# Autodesk Inventor assembly: Vertical Support - with Brackets
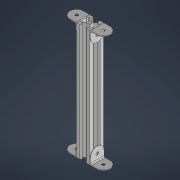
[picture p0: Inventor's stored thumbnail of the model, 180x180]
Saved by Autodesk Inventor 2022 (Build 260153000, 153)
## iProperties
Created: 2023-06-23
Part Number: Vertical Support - with Brackets
Document SubType Name: Assembly
Designer: Ryan Mitcham
Author: Ryan Mitcham
## Documents named in this file (3)
- C:\Users\Gaming\OneDrive\Documents\Inventor\XYZ-Gantry\Support Structure\Vertical Support - with Brackets.iam
- C:\Users\Gaming\OneDrive\Documents\Inventor\XYZ-Gantry\Support Structure\Vertical Support.ipt
- C:\Users\Gaming\OneDrive\Documents\Inventor\XYZ-Gantry\Support Structure\Vertical Support - 90deg Bracket.ipt
## Components (5 placed, 2 different names)
1. Vertical Support:1 — Mate:1, Mate:2, Mate:3, Mate:4, Flush:1, Flush:2, Flush:3, Flush:4, Mate:5, Mate:6, Flush:5, Flush:6, Flush:7, Mate:7, Flush:8
2. Vertical Support - 90deg Bracket:1 — Flush:3, Flush:4, Mate:5
3. Vertical Support - 90deg Bracket:2 — Mate:4, Flush:1, Flush:2
4. Vertical Support - 90deg Bracket:3 — Mate:6, Flush:5, Flush:6
5. Vertical Support - 90deg Bracket:4 — Flush:7, Mate:7, Flush:8
## Relationships (15: Flush 8, Mate 7)
- Mate:1: Vertical Support:1
- Mate:2: Vertical Support:1
- Mate:3: Vertical Support:1
- Mate:4: Vertical Support:1 ↔ Vertical Support - 90deg Bracket:2
- Flush:1: Vertical Support:1 ↔ Vertical Support - 90deg Bracket:2
- Flush:2: Vertical Support:1 ↔ Vertical Support - 90deg Bracket:2
- Flush:3: Vertical Support:1 ↔ Vertical Support - 90deg Bracket:1
- Flush:4: Vertical Support:1 ↔ Vertical Support - 90deg Bracket:1
- Mate:5: Vertical Support:1 ↔ Vertical Support - 90deg Bracket:1
- Mate:6: Vertical Support:1 ↔ Vertical Support - 90deg Bracket:3
- Flush:5: Vertical Support:1 ↔ Vertical Support - 90deg Bracket:3
- Flush:6: Vertical Support:1 ↔ Vertical Support - 90deg Bracket:3
- Flush:7: Vertical Support:1 ↔ Vertical Support - 90deg Bracket:4
- Mate:7: Vertical Support:1 ↔ Vertical Support - 90deg Bracket:4
- Flush:8: Vertical Support:1 ↔ Vertical Support - 90deg Bracket:4
